# Autodesk Inventor assembly: Leg_Right
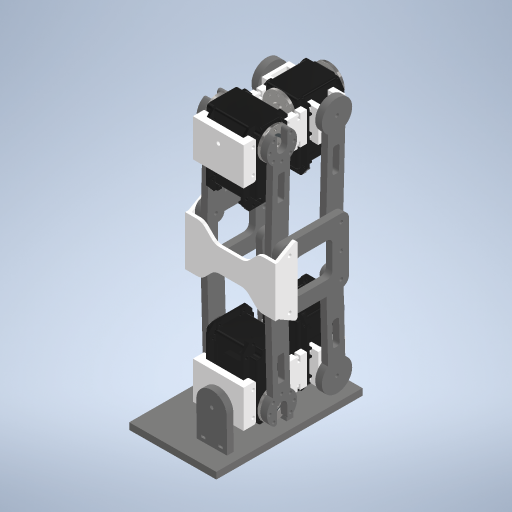
[picture p0: Inventor's stored thumbnail of the model, 512x512]
Saved by Autodesk Inventor 2024.3 (Build 283343000, 343)
## iProperties
Created: 2024-09-18
Part Number: Leg_Right
Document SubType Name: Assembly
Designer: 구지현
Author: 구지현
## Documents named in this file (20)
- C:\Users\구지현\Desktop\19th_intern_kdy_fight_robot\부품\Lower_Body\Leg\Leg_Right.iam
- C:\Users\구지현\Desktop\19th_intern_kdy_fight_robot\부품\Lower_Body\Leg\Back_Ankle.ipt
- C:\Users\구지현\Desktop\19th_intern_kdy_fight_robot\부품\Lower_Body\Leg\Foot_MIR.ipt
- C:\Users\구지현\Desktop\19th_intern_kdy_fight_robot\부품\Lower_Body\Leg\Front_Ankle.ipt
- C:\Users\구지현\Desktop\19th_intern_kdy_fight_robot\부품\Lower_Body\Leg\Knee.ipt
- C:\Users\구지현\Desktop\19th_intern_kdy_fight_robot\부품\Lower_Body\Leg\Knee_Covers.ipt
- C:\Users\구지현\Desktop\19th_intern_kdy_fight_robot\부품\Lower_Body\Leg\Leg_Connection_Parts_Back.ipt
- C:\Users\구지현\Desktop\19th_intern_kdy_fight_robot\부품\Lower_Body\Leg\Leg_Connection_Parts_Front.ipt
- C:\Users\구지현\Desktop\19th_intern_kdy_fight_robot\부품\Lower_Body\Leg\Leg_Foot_Connection_Parts.ipt
- C:\Users\구지현\Desktop\19th_intern_kdy_fight_robot\부품\Lower_Body\Leg\Link_Fixation_Connector.ipt
- C:\Users\구지현\Desktop\19th_intern_kdy_fight_robot\부품\Lower_Body\Leg\Link_Fixation_Connector_MIR.ipt
- Link_Fixation_Connector_left_left.ipt
- C:\Users\구지현\Desktop\19th_intern_kdy_fight_robot\부품\Lower_Body\Leg\Link_Fixation_Connector_MIR_MIR.ipt
- C:\Users\구지현\Desktop\19th_intern_kdy_fight_robot\부품\Lower_Body\Leg\Link_Fixation_Connector_MIR1.ipt
- C:\Users\구지현\Desktop\19th_intern_kdy_fight_robot\부품\Lower_Body\Leg\Vertical_Fixation_Set.iam
- C:\Users\구지현\Desktop\19th_intern_kdy_fight_robot\부품\ROBOTIS(Inventor 2024 ver.)\다이나믹셀\MX-64T+idle.ipt.iam
- C:\Users\구지현\Desktop\19th_intern_kdy_fight_robot\부품\ROBOTIS(Inventor 2024 ver.)\다이나믹셀\MX-106T+idle.ipt.iam
- C:\Users\구지현\Desktop\19th_intern_kdy_fight_robot\부품\ROBOTIS(Inventor 2024 ver.)\혼\64-106Horn.ipt
- MX-64T+idle.ipt
- MX-106T+idle.ipt
## Components (30 placed, 16 different names)
1. Back_Ankle:1 — 플러쉬:1, 각도:1, 삽입:14
2. Foot_MIR:1 — 삽입:13, 삽입:14
3. Front_Ankle:1 — 삽입:11, 플러쉬:1, 각도:1, 삽입:13
4. Knee:1 — 삽입:15, 삽입:18, 플러쉬:6, 플러쉬:7, 삽입:20, 삽입:21, 삽입:25, 삽입:36
5. Knee_Covers:1 — 삽입:20, 삽입:21, 삽입:22, 삽입:23
6. Leg_Connection_Parts_Front:1 — 플러쉬:2, 플러쉬:3, 삽입:15, 플러쉬:4, 각도:2, 메이트:36, 메이트:37
7. Leg_Foot_Connection_Parts:1 — 삽입:11, 플러쉬:18, 메이트:38, 메이트:39
8. Link_Fixation_Connector_left_left:1 — 메이트:17, 메이트:49, 메이트:50, 메이트:51
9. Vertical_Fixation_Set:1 [sub-assembly] — 메이트:40, 메이트:41, 삽입:43, 삽입:44
10. Leg_Connection_Parts_Front:2 — 플러쉬:2, 플러쉬:3, 삽입:17, 플러쉬:5, 각도:3
11. Leg_Connection_Parts_Back:4 — 플러쉬:4, 각도:2, 삽입:18, 플러쉬:8, 메이트:21
12. Leg_Connection_Parts_Back:5 — 플러쉬:5, 각도:3, 삽입:19, 플러쉬:8, 메이트:17
13. Knee:2 — 삽입:17, 플러쉬:6, 플러쉬:7, 삽입:19, 삽입:22, 삽입:23, 삽입:24, 삽입:35
14. Link_Fixation_Connector:2 — 메이트:21
15. Link_Fixation_Connector_MIR1:4 — 메이트:29
16. Leg_Connection_Parts_Front:3 — 플러쉬:11, 플러쉬:12, 삽입:24, 플러쉬:15, 각도:5
17. Leg_Connection_Parts_Front:4 — 플러쉬:11, 플러쉬:12, 삽입:25, 플러쉬:16, 각도:6, 메이트:34, 메이트:35
18. Leg_Connection_Parts_Back:6 — 삽입:36, 플러쉬:16, 플러쉬:17, 각도:6, 메이트:29
19. Leg_Connection_Parts_Back:7 — 삽입:35, 플러쉬:15, 각도:5, 플러쉬:17, 메이트:33
20. Vertical_Fixation_Set:2 [sub-assembly] — 메이트:44, 메이트:45, 삽입:41, 삽입:42
21. Link_Fixation_Connector_MIR_MIR:2 — 메이트:33, 메이트:46, 메이트:47, 메이트:48
22. Leg_Foot_Connection_Parts:3 — 플러쉬:18, 메이트:42, 메이트:43
23. MX-64T+idle.ipt:1 [sub-assembly] — 삽입:40, 삽입:43, 삽입:44, 메이트:49, 메이트:50, 메이트:51
24. MX-64T+idle.ipt:2 [sub-assembly] — 삽입:39, 삽입:41, 삽입:42, 메이트:46, 메이트:47, 메이트:48
25. MX-106T+idle.ipt:1 [sub-assembly] — 삽입:38, 플러쉬:19, 각도:7, 메이트:42, 메이트:43, 메이트:44, 메이트:45
26. MX-106T+idle.ipt:2 [sub-assembly] — 삽입:37, 메이트:38, 메이트:39, 메이트:40, 메이트:41, 플러쉬:19, 각도:7
27. 64-106Horn:1 — 삽입:39
28. 64-106Horn:2 — 메이트:36, 메이트:37, 삽입:37
29. 64-106Horn:3 — 삽입:40
30. 64-106Horn:4 — 메이트:34, 메이트:35, 삽입:38
## Relationships (66: Insert 23, Mate 22, Flush 15, Angle 6)
- 삽입:11 [Insert]: Front_Ankle:1 ↔ Leg_Foot_Connection_Parts:1
- 플러쉬:1 [Flush]: Back_Ankle:1 ↔ Front_Ankle:1
- 각도:1 [Angle] (0 deg): Back_Ankle:1 ↔ Front_Ankle:1
- 삽입:13 [Insert]: Foot_MIR:1 ↔ Front_Ankle:1
- 삽입:14 [Insert]: Back_Ankle:1 ↔ Foot_MIR:1
- 플러쉬:2 [Flush]: Leg_Connection_Parts_Front:1 ↔ Leg_Connection_Parts_Front:2
- 플러쉬:3 [Flush]: Leg_Connection_Parts_Front:1 ↔ Leg_Connection_Parts_Front:2
- 삽입:15 [Insert]: Knee:1 ↔ Leg_Connection_Parts_Front:1
- 삽입:17 [Insert]: Leg_Connection_Parts_Front:2 ↔ Knee:2
- 플러쉬:4 [Flush]: Leg_Connection_Parts_Front:1 ↔ Leg_Connection_Parts_Back:4
- 각도:2 [Angle] (0 deg): Leg_Connection_Parts_Front:1 ↔ Leg_Connection_Parts_Back:4
- 삽입:18 [Insert]: Knee:1 ↔ Leg_Connection_Parts_Back:4
- 플러쉬:5 [Flush]: Leg_Connection_Parts_Front:2 ↔ Leg_Connection_Parts_Back:5
- 각도:3 [Angle] (0 deg): Leg_Connection_Parts_Front:2 ↔ Leg_Connection_Parts_Back:5
- 플러쉬:6 [Flush]: Knee:1 ↔ Knee:2
- 플러쉬:7 [Flush]: Knee:1 ↔ Knee:2
- 삽입:19 [Insert]: Leg_Connection_Parts_Back:5 ↔ Knee:2
- 플러쉬:8 [Flush]: Leg_Connection_Parts_Back:4 ↔ Leg_Connection_Parts_Back:5
- 메이트:17 [Mate]: Link_Fixation_Connector_left_left:1 ↔ Leg_Connection_Parts_Back:5
- 메이트:21 [Mate]: Leg_Connection_Parts_Back:4 ↔ Link_Fixation_Connector:2
- 삽입:20 [Insert]: Knee:1 ↔ Knee_Covers:1
- 삽입:21 [Insert]: Knee:1 ↔ Knee_Covers:1
- 삽입:22 [Insert]: Knee_Covers:1 ↔ Knee:2
- 삽입:23 [Insert]: Knee_Covers:1 ↔ Knee:2
- 플러쉬:11 [Flush]: Leg_Connection_Parts_Front:3 ↔ Leg_Connection_Parts_Front:4
- 플러쉬:12 [Flush]: Leg_Connection_Parts_Front:3 ↔ Leg_Connection_Parts_Front:4
- 삽입:24 [Insert]: Knee:2 ↔ Leg_Connection_Parts_Front:3
- 삽입:25 [Insert]: Knee:1 ↔ Leg_Connection_Parts_Front:4
- 삽입:35 [Insert]: Knee:2 ↔ Leg_Connection_Parts_Back:7
- 플러쉬:15 [Flush]: Leg_Connection_Parts_Front:3 ↔ Leg_Connection_Parts_Back:7
- 각도:5 [Angle] (0 deg): Leg_Connection_Parts_Front:3 ↔ Leg_Connection_Parts_Back:7
- 삽입:36 [Insert]: Knee:1 ↔ Leg_Connection_Parts_Back:6
- 플러쉬:16 [Flush]: Leg_Connection_Parts_Front:4 ↔ Leg_Connection_Parts_Back:6
- 플러쉬:17 [Flush]: Leg_Connection_Parts_Back:6 ↔ Leg_Connection_Parts_Back:7
- 각도:6 [Angle] (0 deg): Leg_Connection_Parts_Front:4 ↔ Leg_Connection_Parts_Back:6
- 메이트:29 [Mate]: Link_Fixation_Connector_MIR1:4 ↔ Leg_Connection_Parts_Back:6
- 메이트:33 [Mate]: Leg_Connection_Parts_Back:7 ↔ Link_Fixation_Connector_MIR_MIR:2
- 플러쉬:18 [Flush]: Leg_Foot_Connection_Parts:1 ↔ Leg_Foot_Connection_Parts:3
- 메이트:34 [Mate]: Leg_Connection_Parts_Front:4 ↔ 64-106Horn:4
- 메이트:35 [Mate]: Leg_Connection_Parts_Front:4 ↔ 64-106Horn:4
- 메이트:36 [Mate]: Leg_Connection_Parts_Front:1 ↔ 64-106Horn:2
- 메이트:37 [Mate]: Leg_Connection_Parts_Front:1 ↔ 64-106Horn:2
- 삽입:37 [Insert]: MX-106T+idle.ipt:2 ↔ 64-106Horn:2
- 메이트:38 [Mate]: Leg_Foot_Connection_Parts:1 ↔ MX-106T+idle.ipt:2
- 메이트:39 [Mate]: Leg_Foot_Connection_Parts:1 ↔ MX-106T+idle.ipt:2
- 메이트:40 [Mate]: Vertical_Fixation_Set:1 ↔ MX-106T+idle.ipt:2
- 메이트:41 [Mate]: Vertical_Fixation_Set:1 ↔ MX-106T+idle.ipt:2
- 삽입:38 [Insert]: MX-106T+idle.ipt:1 ↔ 64-106Horn:4
- 플러쉬:19 [Flush]: MX-106T+idle.ipt:1 ↔ MX-106T+idle.ipt:2
- 각도:7 [Angle] (0 deg): MX-106T+idle.ipt:1 ↔ MX-106T+idle.ipt:2
- 메이트:42 [Mate]: Leg_Foot_Connection_Parts:3 ↔ MX-106T+idle.ipt:1
- 메이트:43 [Mate]: Leg_Foot_Connection_Parts:3 ↔ MX-106T+idle.ipt:1
- 메이트:44 [Mate]: Vertical_Fixation_Set:2 ↔ MX-106T+idle.ipt:1
- 메이트:45 [Mate]: Vertical_Fixation_Set:2 ↔ MX-106T+idle.ipt:1
- 삽입:39 [Insert]: MX-64T+idle.ipt:2 ↔ 64-106Horn:1
- 삽입:40 [Insert]: MX-64T+idle.ipt:1 ↔ 64-106Horn:3
- 삽입:41 [Insert]: Vertical_Fixation_Set:2 ↔ MX-64T+idle.ipt:2
- 삽입:42 [Insert]: Vertical_Fixation_Set:2 ↔ MX-64T+idle.ipt:2
- 메이트:46 [Mate]: Link_Fixation_Connector_MIR_MIR:2 ↔ MX-64T+idle.ipt:2
- 메이트:47 [Mate]: Link_Fixation_Connector_MIR_MIR:2 ↔ MX-64T+idle.ipt:2
- 메이트:48 [Mate] (0.1 mm): Link_Fixation_Connector_MIR_MIR:2 ↔ MX-64T+idle.ipt:2
- 삽입:43 [Insert]: Vertical_Fixation_Set:1 ↔ MX-64T+idle.ipt:1
- 삽입:44 [Insert]: Vertical_Fixation_Set:1 ↔ MX-64T+idle.ipt:1
- 메이트:49 [Mate]: Link_Fixation_Connector_left_left:1 ↔ MX-64T+idle.ipt:1
- 메이트:50 [Mate]: Link_Fixation_Connector_left_left:1 ↔ MX-64T+idle.ipt:1
- 메이트:51 [Mate] (0.1 mm): Link_Fixation_Connector_left_left:1 ↔ MX-64T+idle.ipt:1
